# Autodesk Inventor assembly: Piezas3D
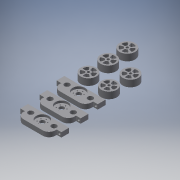
[picture p0: Inventor's stored thumbnail of the model, 180x180]
Saved by Autodesk Inventor 2017 (Build 210142000, 142)
## iProperties
Created: 2017-05-03
Part Number: Piezas3D
Document SubType Name: Assembly
Designer: ANDRES
Author: ANDRES
## Documents named in this file (3)
- D:\MIS COSAS\Drive\Publica\UCABBOTS2017\Laberinto\Diseño Mecanico\Impresiones3D\Piezas3D.iam
- D:\MIS COSAS\Drive\Publica\UCABBOTS2017\Laberinto\Diseño Mecanico\Base_Motor_acrilico_15.ipt
- D:\MIS COSAS\Drive\Publica\UCABBOTS2017\Laberinto\Diseño Mecanico\Rueda_Rin_Final.ipt
## Components (8 placed, 2 different names)
1. Base_Motor_acrilico_15:1 — Mate:2
2. Rueda_Rin_Final:1 — Mate:3
3. Base_Motor_acrilico_15:2 — Mate:1
4. Rueda_Rin_Final:2 — Mate:6
5. Rueda_Rin_Final:3 — Mate:5
6. Rueda_Rin_Final:4 — Mate:4
7. Base_Motor_acrilico_15:3 — Mate:7
8. Rueda_Rin_Final:5 — Mate:8
## Relationships (8: Mate 8)
- Mate:1: Base_Motor_acrilico_15:2
- Mate:2: Base_Motor_acrilico_15:1
- Mate:3: Rueda_Rin_Final:1
- Mate:4: Rueda_Rin_Final:4
- Mate:5: Rueda_Rin_Final:3
- Mate:6: Rueda_Rin_Final:2
- Mate:7: Base_Motor_acrilico_15:3
- Mate:8: Rueda_Rin_Final:5
